# Autodesk Inventor assembly: MGN7H-rail-100
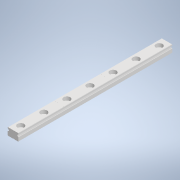
[picture p0: Inventor's stored thumbnail of the model, 180x180]
Saved by Autodesk Inventor 2022 (Build 260153000, 153)
## iProperties
Created: 2021-11-24
Part Number: MGN7H-rail-100
Document SubType Name: Assembly
Designer: yuto6
Author: yuto6
## Documents named in this file (2)
- C:\Users\yuto6\Documents\My3DPrinter\Downloads\MGN7H-rail-100.iam
- C:\Users\yuto6\Documents\My3DPrinter\Downloads\MANIFOLD_SOLID_BREP_80.ipt
## Components (3 placed, 1 different names)
1. MANIFOLD_SOLID_BREP_80:1 — メイト:1, フラッシュ:1, メイト:2, フラッシュ:2, フラッシュ:3, フラッシュ:4
2. MANIFOLD_SOLID_BREP_80:2 — メイト:1, フラッシュ:1, フラッシュ:3
3. MANIFOLD_SOLID_BREP_80:3 — メイト:2, フラッシュ:2, フラッシュ:4
## Relationships (6: Flush 4, Mate 2)
- メイト:1 [Mate]: MANIFOLD_SOLID_BREP_80:1 ↔ MANIFOLD_SOLID_BREP_80:2
- フラッシュ:1 [Flush]: MANIFOLD_SOLID_BREP_80:1 ↔ MANIFOLD_SOLID_BREP_80:2
- メイト:2 [Mate]: MANIFOLD_SOLID_BREP_80:1 ↔ MANIFOLD_SOLID_BREP_80:3
- フラッシュ:2 [Flush]: MANIFOLD_SOLID_BREP_80:1 ↔ MANIFOLD_SOLID_BREP_80:3
- フラッシュ:3 [Flush]: MANIFOLD_SOLID_BREP_80:1 ↔ MANIFOLD_SOLID_BREP_80:2
- フラッシュ:4 [Flush]: MANIFOLD_SOLID_BREP_80:1 ↔ MANIFOLD_SOLID_BREP_80:3
